# Autodesk Inventor assembly: Assembly air purification and monitoring
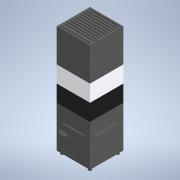
[picture p0: Inventor's stored thumbnail of the model, 180x180]
Saved by Autodesk Inventor 2021 (Build 250183000, 183)
## iProperties
Created: 2025-07-05
Part Number: Assembly air purification and monitoring
Document SubType Name: Assembly
Designer: Apanzia
Author: Apanzia
## Documents named in this file (8)
- C:\Users\Apanzia\Documents\Assembly air purification and monitoring.iam
- C:\Users\Apanzia\Documents\base and electronics hub.ipt
- C:\Users\Apanzia\Documents\lid.ipt
- C:\Users\Apanzia\Documents\UV chamber and outlet.ipt
- C:\Users\Apanzia\Documents\carbon particle filter.ipt
- C:\Users\Apanzia\Documents\HEPA air filter.ipt
- C:\Users\Apanzia\Documents\fan duct.ipt
- C:\Users\Apanzia\Documents\fan duct1.ipt
## Components (7 placed, 7 different names)
1. base and electronics hub:1 — Mate:1, Flush:1, Flush:2, Flush:3, Flush:4
2. lid:1 — Mate:1, Flush:1, Flush:2, Mate:2
3. UV chamber and outlet:1 — Mate:2, Flush:3, Flush:4, Mate:3, Flush:5, Flush:6
4. carbon particle filter:1 — Mate:3, Flush:5, Flush:6, Mate:4, Flush:7
5. HEPA air filter:1 — Mate:4, Flush:7, Mate:5, Flush:8, Flush:9
6. fan duct:1 — Mate:5, Flush:8, Flush:9, Mate:6, Flush:10
7. fan duct1:1 — Mate:6, Flush:10
## Relationships (16: Flush 10, Mate 6)
- Mate:1: base and electronics hub:1 ↔ lid:1
- Flush:1: base and electronics hub:1 ↔ lid:1
- Flush:2: base and electronics hub:1 ↔ lid:1
- Mate:2: lid:1 ↔ UV chamber and outlet:1
- Flush:3: base and electronics hub:1 ↔ UV chamber and outlet:1
- Flush:4: base and electronics hub:1 ↔ UV chamber and outlet:1
- Mate:3: UV chamber and outlet:1 ↔ carbon particle filter:1
- Flush:5: UV chamber and outlet:1 ↔ carbon particle filter:1
- Flush:6: UV chamber and outlet:1 ↔ carbon particle filter:1
- Mate:4: carbon particle filter:1 ↔ HEPA air filter:1
- Flush:7: carbon particle filter:1 ↔ HEPA air filter:1
- Mate:5: HEPA air filter:1 ↔ fan duct:1
- Flush:8: HEPA air filter:1 ↔ fan duct:1
- Flush:9: HEPA air filter:1 ↔ fan duct:1
- Mate:6: fan duct:1 ↔ fan duct1:1
- Flush:10: fan duct:1 ↔ fan duct1:1
